# Autodesk Inventor assembly: Y Axis Assembly
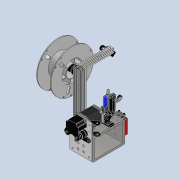
[picture p0: Inventor's stored thumbnail of the model, 180x180]
Saved by Autodesk Inventor 2022 (Build 260153000, 153)
## iProperties
Created: 2021-10-17
Part Number: Y Axis Assembly
Document SubType Name: Assembly
Designer: Coy
Author: Coy
## Documents named in this file (25)
- H:\3D Files\Project 3D Models\Breakfast Maker 2000\Assemblys\Y Axis Assembly.iam
- H:\3D Files\Project 3D Models\Breakfast Maker 2000\Machined Parts\4in x 6in Steel Rectangular Tubing 4in long Machined.ipt
- H:\3D Files\Project 3D Models\Breakfast Maker 2000\Machined Parts\X Axis Belt Motor Inside Frame Machined.ipt
- H:\3D Files\Project 3D Models\Breakfast Maker 2000\Motors\Nema 23 76.5mm Stepper Motor.ipt
- H:\3D Files\Project 3D Models\Breakfast Maker 2000\Pullys\M6.35 24Tooth 15mm Deep 3M Timing Pulley.ipt
- H:\3D Files\Project 3D Models\Breakfast Maker 2000\3D Printed Parts\X Axis Pully Support.ipt
- H:\3D Files\Project 3D Models\Breakfast Maker 2000\Shafts and Rods\M5 60mm Threaded Rod.ipt
- H:\3D Files\Project 3D Models\Breakfast Maker 2000\Pullys\8mm ID 15mm Deep Idler Pully.ipt
- H:\3D Files\Project 3D Models\Breakfast Maker 2000\Bearings\5mm ID 8mm OD 2.5mm Deep Roller Bearing (2021_08_15 23_37_01 UTC).ipt
- H:\3D Files\Project 3D Models\Breakfast Maker 2000\Nuts and Bolts\M5 Nut Silver.ipt
- H:\3D Files\Project 3D Models\Breakfast Maker 2000\3D Printed Parts\Idler Pully Spacer X Axis 3mm.ipt
- H:\3D Files\Project 3D Models\Breakfast Maker 2000\3D Printed Parts\Idler Pully Spacer X Axis 7mm.ipt
- H:\3D Files\Project 3D Models\Breakfast Maker 2000\Linear Actuators\Z Axis Statonary Block.ipt
- H:\3D Files\Project 3D Models\Breakfast Maker 2000\Sensors\High Voltage Limit Switch\High Voltage Limit Switch.ipt
- H:\3D Files\Project 3D Models\Breakfast Maker 2000\Sensors\High Voltage Limit Switch\High Voltage Limit Switch Arm.ipt
- H:\3D Files\Project 3D Models\Breakfast Maker 2000\Sensors\High Voltage Limit Switch\High Voltage Limit Switch Arm Coupler.ipt
- H:\3D Files\Project 3D Models\Breakfast Maker 2000\3D Printed Parts\Y Axis Limit Switch and Drag Chain Mount.ipt
- H:\3D Files\Project 3D Models\Breakfast Maker 2000\3D Printed Parts\Y Axis Limit Switch Trigger.ipt
- H:\3D Files\Project 3D Models\Breakfast Maker 2000\3D Printed Parts\Y Axis Drag Chain Mount Bolted.ipt
- H:\3D Files\Project 3D Models\Breakfast Maker 2000\2020 Extrusion 90deg 2Hole Aluminum Bracket.ipt
- H:\3D Files\Project 3D Models\Breakfast Maker 2000\Aluminum Extrusion\2040\2040x200 silver profile.ipt
- H:\3D Files\Project 3D Models\Breakfast Maker 2000\Aluminum Extrusion\2020\20mm X 20mm X 150mm aluminium profile v slot.ipt
- H:\3D Files\Project 3D Models\Breakfast Maker 2000\Filament Spool Holder.ipt
- H:\3D Files\Project 3D Models\Breakfast Maker 2000\Overture Filament Spool v1.ipt
- H:\3D Files\Project 3D Models\Breakfast Maker 2000\90 deg Shelf 4 Hole Bracket.ipt
## Components (35 placed, 24 different names)
1. 4in x 6in Steel Rectangular Tubing 4in long Machined:1 — Mate:1, Mate:2, Mate:3, Mate:36, Mate:37, Mate:38, Mate:44, Mate:45, Mate:46, Mate:56, Flush:10, Flush:12
2. X Axis Belt Motor Inside Frame Machined:1 — Mate:1, Mate:2, Mate:3, Mate:5, Mate:6, Mate:7, Mate:10, Mate:11, Mate:12, Mate:13, Mate:14, Mate:32, Mate:33, Mate:50, Mate:51, Mate:52, Mate:53, Mate:54, Mate:55
3. Nema 23 76.5mm Stepper Motor:1 — Mate:5, Mate:6, Mate:7, Mate:8, Mate:9, Mate:25, Mate:26
4. M6.35 24Tooth 15mm Deep 3M Timing Pulley:1 — Mate:8, Mate:9, Flush:7, Flush:8
5. X Axis Pully Support:1 — Mate:10, Mate:11, Mate:12, Flush:1, Mate:27, Mate:34, Mate:35
6. M5 60mm Threaded Rod:1 — Mate:14, Flush:2, Mate:19, Mate:21, Mate:24, Mate:29, Mate:31
7. M5 60mm Threaded Rod:2 — Mate:13, Flush:1, Flush:2, Mate:20, Mate:22, Mate:23, Mate:28, Mate:30
8. 8mm ID 15mm Deep Idler Pully:1 — Mate:16, Flush:4, Mate:18, Flush:6, Flush:7
9. 8mm ID 15mm Deep Idler Pully:2 — Mate:15, Flush:3, Mate:17, Flush:5, Flush:8
10. 5mm ID 8mm OD 2.5mm Deep Roller Bearing (2021_08_15 23_37_01 UTC):1 — Mate:18, Flush:6, Mate:20
11. 5mm ID 8mm OD 2.5mm Deep Roller Bearing (2021_08_15 23_37_01 UTC):2 — Mate:15, Flush:3
12. 5mm ID 8mm OD 2.5mm Deep Roller Bearing (2021_08_15 23_37_01 UTC):3 — Mate:17, Flush:5, Mate:19
13. 5mm ID 8mm OD 2.5mm Deep Roller Bearing (2021_08_15 23_37_01 UTC):4 — Mate:16, Flush:4
14. M5 Nut Silver:1 — Mate:22, Mate:27, Flush:9
15. M5 Nut Silver:2 — Mate:23, Mate:26
16. M5 Nut Silver:3 — Mate:21, Flush:9
17. M5 Nut Silver:4 — Mate:24, Mate:25
18. Idler Pully Spacer X Axis 3mm:1 — Mate:31, Mate:32
19. Idler Pully Spacer X Axis 3mm:2 — Mate:30, Mate:33
20. Idler Pully Spacer X Axis 7mm:1 — Mate:29, Mate:35
21. Idler Pully Spacer X Axis 7mm:2 — Mate:28, Mate:34
22. Z Axis Statonary Block:1 — Mate:36, Mate:37, Mate:38
23. High Voltage Limit Switch:1 — Mate:39, Mate:40, Mate:47, Mate:48, Mate:49
24. High Voltage Limit Switch Arm:1 — Mate:41, Mate:42
25. High Voltage Limit Switch Arm Coupler:1 — Mate:39, Mate:40, Mate:41, Mate:42
26. Y Axis Limit Switch and Drag Chain Mount:1 — Mate:44, Mate:45, Mate:46, Mate:47, Mate:48, Mate:49, Mate:57
27. Y Axis Limit Switch Trigger:1 — Mate:50, Mate:51, Mate:52
28. Y Axis Drag Chain Mount Bolted:1 — Mate:53, Mate:54, Mate:55
29. 2020 Extrusion 90deg 2Hole Aluminum Bracket:1 — Mate:56, Flush:10, Mate:57, Mate:58, Flush:11
30. 2040x200 silver profile:1 — Mate:58, Flush:11, Flush:12, Mate:59, Flush:13, Mate:60, Flush:14, Flush:15, Mate:62, Tangent:2, Tangent:3
31. 2020 Extrusion 90deg 2Hole Aluminum Bracket:2 — Mate:59, Flush:13, Mate:61
32. 20mm X 20mm X 150mm aluminium profile v slot:1 — Mate:60, Flush:14, Flush:15, Mate:61, Mate:65, Flush:16, Flush:17, Mate:67, Angle:1, Angle:2
33. Filament Spool Holder:1 — Mate:62, Tangent:2, Tangent:3, Mate:63, Mate:64
34. Overture Filament Spool v1:1 — Mate:63, Mate:64
35. 90 deg Shelf 4 Hole Bracket:1 — Mate:65, Mate:70, Angle:2
## Relationships (89: Mate 68, Flush 17, Tangent 2, Angle 2)
- Mate:1: 4in x 6in Steel Rectangular Tubing 4in long Machined:1 ↔ X Axis Belt Motor Inside Frame Machined:1
- Mate:2: 4in x 6in Steel Rectangular Tubing 4in long Machined:1 ↔ X Axis Belt Motor Inside Frame Machined:1
- Mate:3: 4in x 6in Steel Rectangular Tubing 4in long Machined:1 ↔ X Axis Belt Motor Inside Frame Machined:1
- Mate:5: X Axis Belt Motor Inside Frame Machined:1 ↔ Nema 23 76.5mm Stepper Motor:1
- Mate:6: X Axis Belt Motor Inside Frame Machined:1 ↔ Nema 23 76.5mm Stepper Motor:1
- Mate:7: X Axis Belt Motor Inside Frame Machined:1 ↔ Nema 23 76.5mm Stepper Motor:1
- Mate:8: Nema 23 76.5mm Stepper Motor:1 ↔ M6.35 24Tooth 15mm Deep 3M Timing Pulley:1
- Mate:9 (0.15 mm): Nema 23 76.5mm Stepper Motor:1 ↔ M6.35 24Tooth 15mm Deep 3M Timing Pulley:1
- Mate:10: X Axis Belt Motor Inside Frame Machined:1 ↔ X Axis Pully Support:1
- Mate:11: X Axis Belt Motor Inside Frame Machined:1 ↔ X Axis Pully Support:1
- Mate:12: X Axis Belt Motor Inside Frame Machined:1 ↔ X Axis Pully Support:1
- Mate:13: X Axis Belt Motor Inside Frame Machined:1 ↔ M5 60mm Threaded Rod:2
- Mate:14: X Axis Belt Motor Inside Frame Machined:1 ↔ M5 60mm Threaded Rod:1
- Flush:1 (-5 mm): X Axis Pully Support:1 ↔ M5 60mm Threaded Rod:2
- Flush:2: M5 60mm Threaded Rod:1 ↔ M5 60mm Threaded Rod:2
- Mate:15: 8mm ID 15mm Deep Idler Pully:2 ↔ 5mm ID 8mm OD 2.5mm Deep Roller Bearing (2021_08_15 23_37_01 UTC):2
- Flush:3: 8mm ID 15mm Deep Idler Pully:2 ↔ 5mm ID 8mm OD 2.5mm Deep Roller Bearing (2021_08_15 23_37_01 UTC):2
- Mate:16: 8mm ID 15mm Deep Idler Pully:1 ↔ 5mm ID 8mm OD 2.5mm Deep Roller Bearing (2021_08_15 23_37_01 UTC):4
- Flush:4: 8mm ID 15mm Deep Idler Pully:1 ↔ 5mm ID 8mm OD 2.5mm Deep Roller Bearing (2021_08_15 23_37_01 UTC):4
- Mate:17: 8mm ID 15mm Deep Idler Pully:2 ↔ 5mm ID 8mm OD 2.5mm Deep Roller Bearing (2021_08_15 23_37_01 UTC):3
- Flush:5: 8mm ID 15mm Deep Idler Pully:2 ↔ 5mm ID 8mm OD 2.5mm Deep Roller Bearing (2021_08_15 23_37_01 UTC):3
- Mate:18: 8mm ID 15mm Deep Idler Pully:1 ↔ 5mm ID 8mm OD 2.5mm Deep Roller Bearing (2021_08_15 23_37_01 UTC):1
- Flush:6: 8mm ID 15mm Deep Idler Pully:1 ↔ 5mm ID 8mm OD 2.5mm Deep Roller Bearing (2021_08_15 23_37_01 UTC):1
- Mate:19: M5 60mm Threaded Rod:1 ↔ 5mm ID 8mm OD 2.5mm Deep Roller Bearing (2021_08_15 23_37_01 UTC):3
- Mate:20: M5 60mm Threaded Rod:2 ↔ 5mm ID 8mm OD 2.5mm Deep Roller Bearing (2021_08_15 23_37_01 UTC):1
- Flush:7: M6.35 24Tooth 15mm Deep 3M Timing Pulley:1 ↔ 8mm ID 15mm Deep Idler Pully:1
- Flush:8: M6.35 24Tooth 15mm Deep 3M Timing Pulley:1 ↔ 8mm ID 15mm Deep Idler Pully:2
- Mate:21: M5 60mm Threaded Rod:1 ↔ M5 Nut Silver:3
- Mate:22: M5 60mm Threaded Rod:2 ↔ M5 Nut Silver:1
- Mate:23: M5 60mm Threaded Rod:2 ↔ M5 Nut Silver:2
- Mate:24: M5 60mm Threaded Rod:1 ↔ M5 Nut Silver:4
- Mate:25: Nema 23 76.5mm Stepper Motor:1 ↔ M5 Nut Silver:4
- Mate:26: Nema 23 76.5mm Stepper Motor:1 ↔ M5 Nut Silver:2
- Mate:27: X Axis Pully Support:1 ↔ M5 Nut Silver:1
- Flush:9: M5 Nut Silver:1 ↔ M5 Nut Silver:3
- Mate:28: M5 60mm Threaded Rod:2 ↔ Idler Pully Spacer X Axis 7mm:2
- Mate:29: M5 60mm Threaded Rod:1 ↔ Idler Pully Spacer X Axis 7mm:1
- Mate:30: M5 60mm Threaded Rod:2 ↔ Idler Pully Spacer X Axis 3mm:2
- Mate:31: M5 60mm Threaded Rod:1 ↔ Idler Pully Spacer X Axis 3mm:1
- Mate:32: X Axis Belt Motor Inside Frame Machined:1 ↔ Idler Pully Spacer X Axis 3mm:1
- Mate:33: X Axis Belt Motor Inside Frame Machined:1 ↔ Idler Pully Spacer X Axis 3mm:2
- Mate:34: X Axis Pully Support:1 ↔ Idler Pully Spacer X Axis 7mm:2
- Mate:35: X Axis Pully Support:1 ↔ Idler Pully Spacer X Axis 7mm:1
- Mate:36: 4in x 6in Steel Rectangular Tubing 4in long Machined:1 ↔ Z Axis Statonary Block:1
- Mate:37: 4in x 6in Steel Rectangular Tubing 4in long Machined:1 ↔ Z Axis Statonary Block:1
- Mate:38: 4in x 6in Steel Rectangular Tubing 4in long Machined:1 ↔ Z Axis Statonary Block:1
- Mate:39: High Voltage Limit Switch:1 ↔ High Voltage Limit Switch Arm Coupler:1
- Mate:40 (1.5 mm): High Voltage Limit Switch:1 ↔ High Voltage Limit Switch Arm Coupler:1
- Mate:41: High Voltage Limit Switch Arm:1 ↔ High Voltage Limit Switch Arm Coupler:1
- Mate:42: High Voltage Limit Switch Arm:1 ↔ High Voltage Limit Switch Arm Coupler:1
- Mate:44: 4in x 6in Steel Rectangular Tubing 4in long Machined:1 ↔ Y Axis Limit Switch and Drag Chain Mount:1
- Mate:45: 4in x 6in Steel Rectangular Tubing 4in long Machined:1 ↔ Y Axis Limit Switch and Drag Chain Mount:1
- Mate:46: 4in x 6in Steel Rectangular Tubing 4in long Machined:1 ↔ Y Axis Limit Switch and Drag Chain Mount:1
- Mate:47: High Voltage Limit Switch:1 ↔ Y Axis Limit Switch and Drag Chain Mount:1
- Mate:48: High Voltage Limit Switch:1 ↔ Y Axis Limit Switch and Drag Chain Mount:1
- Mate:49: High Voltage Limit Switch:1 ↔ Y Axis Limit Switch and Drag Chain Mount:1
- Mate:50: X Axis Belt Motor Inside Frame Machined:1 ↔ Y Axis Limit Switch Trigger:1
- Mate:51: X Axis Belt Motor Inside Frame Machined:1 ↔ Y Axis Limit Switch Trigger:1
- Mate:52: X Axis Belt Motor Inside Frame Machined:1 ↔ Y Axis Limit Switch Trigger:1
- Mate:53: X Axis Belt Motor Inside Frame Machined:1 ↔ Y Axis Drag Chain Mount Bolted:1
- Mate:54: X Axis Belt Motor Inside Frame Machined:1 ↔ Y Axis Drag Chain Mount Bolted:1
- Mate:55: X Axis Belt Motor Inside Frame Machined:1 ↔ Y Axis Drag Chain Mount Bolted:1
- Mate:56: 4in x 6in Steel Rectangular Tubing 4in long Machined:1 ↔ 2020 Extrusion 90deg 2Hole Aluminum Bracket:1
- Flush:10: 4in x 6in Steel Rectangular Tubing 4in long Machined:1 ↔ 2020 Extrusion 90deg 2Hole Aluminum Bracket:1
- Mate:57 (9 mm): Y Axis Limit Switch and Drag Chain Mount:1 ↔ 2020 Extrusion 90deg 2Hole Aluminum Bracket:1
- Mate:58: 2020 Extrusion 90deg 2Hole Aluminum Bracket:1 ↔ 2040x200 silver profile:1
- Flush:11 (-1.5 mm): 2020 Extrusion 90deg 2Hole Aluminum Bracket:1 ↔ 2040x200 silver profile:1
- Flush:12: 4in x 6in Steel Rectangular Tubing 4in long Machined:1 ↔ 2040x200 silver profile:1
- Mate:59: 2040x200 silver profile:1 ↔ 2020 Extrusion 90deg 2Hole Aluminum Bracket:2
- Flush:13 (1.5 mm): 2040x200 silver profile:1 ↔ 2020 Extrusion 90deg 2Hole Aluminum Bracket:2
- Mate:60: 2040x200 silver profile:1 ↔ 20mm X 20mm X 150mm aluminium profile v slot:1
- Flush:14: 2040x200 silver profile:1 ↔ 20mm X 20mm X 150mm aluminium profile v slot:1
- Flush:15: 2040x200 silver profile:1 ↔ 20mm X 20mm X 150mm aluminium profile v slot:1
- Mate:61: 2020 Extrusion 90deg 2Hole Aluminum Bracket:2 ↔ 20mm X 20mm X 150mm aluminium profile v slot:1
- Mate:62: 2040x200 silver profile:1 ↔ Filament Spool Holder:1
- Tangent:2: 2040x200 silver profile:1 ↔ Filament Spool Holder:1
- Tangent:3 (-8 mm): 2040x200 silver profile:1 ↔ Filament Spool Holder:1
- Mate:63 (12 mm): Filament Spool Holder:1 ↔ Overture Filament Spool v1:1
- Mate:64 (10 mm): Filament Spool Holder:1 ↔ Overture Filament Spool v1:1
- Mate:65: 20mm X 20mm X 150mm aluminium profile v slot:1 ↔ 90 deg Shelf 4 Hole Bracket:1
- Flush:16 (-10 mm): 20mm X 20mm X 150mm aluminium profile v slot:1
- Flush:17 (-10 mm): 20mm X 20mm X 150mm aluminium profile v slot:1
- Mate:66
- Mate:67: 20mm X 20mm X 150mm aluminium profile v slot:1
- Mate:68
- Mate:69
- Angle:1 (0 deg): 20mm X 20mm X 150mm aluminium profile v slot:1
- Mate:70: 90 deg Shelf 4 Hole Bracket:1
- Angle:2 (50 deg): 20mm X 20mm X 150mm aluminium profile v slot:1 ↔ 90 deg Shelf 4 Hole Bracket:1
